# Autodesk Inventor assembly: Overview
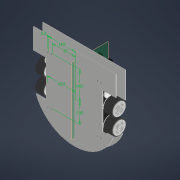
[picture p0: Inventor's stored thumbnail of the model, 180x180]
Saved by Autodesk Inventor 2022 (Build 260153000, 153)
## iProperties
Created: 2021-10-05
Part Number: Overview
Document SubType Name: Assembly
Designer: shiok
Author: shiok
## Documents named in this file (5)
- C:\Users\shiok\Documents\GitHub\murakumo\inventor\Overview.iam
- C:\Users\shiok\Documents\GitHub\murakumo\inventor\flame.ipt
- C:\Users\shiok\Documents\GitHub\murakumo\inventor\Motor.iam
- C:\Users\shiok\Documents\GitHub\murakumo\inventor\Motor_MIR1.iam
- C:\Users\shiok\Documents\GitHub\murakumo\inventor\top.ipt
## Components (4 placed, 4 different names)
1. flame:1 — 挿入:1, 挿入:2
2. Motor:1 [sub-assembly] — フラッシュ:1, メイト:2, 挿入:1
3. Motor_MIR1:1 [sub-assembly] — メイト:1, フラッシュ:2, メイト:3, 挿入:2
4. top:1 — メイト:2, フラッシュ:2, メイト:3
## Relationships (7: Mate 3, Flush 2, Insert 2)
- フラッシュ:1 [Flush] (-42.5 mm): Motor:1
- メイト:1 [Mate] (-42.5 mm): Motor_MIR1:1
- メイト:2 [Mate]: Motor:1 ↔ top:1
- フラッシュ:2 [Flush]: Motor_MIR1:1 ↔ top:1
- メイト:3 [Mate]: Motor_MIR1:1 ↔ top:1
- 挿入:1 [Insert]: flame:1 ↔ Motor:1
- 挿入:2 [Insert]: flame:1 ↔ Motor_MIR1:1
